# Autodesk Inventor assembly: Tesla_Coul
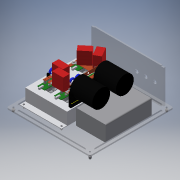
[picture p0: Inventor's stored thumbnail of the model, 180x180]
Saved by Autodesk Inventor 2016 (Build 200138000, 138)
## iProperties
Created: 2018-04-27
Part Number: Tesla_Coul
Document SubType Name: Assembly
Designer: Phil Erle
Author: Phil Erle
## Documents named in this file (43)
- C:\Users\Phil Erle\Desktop\Adrastea\Tesla_Coil.iam
- C:\Users\Phil Erle\Desktop\Adrastea\primary_holder.ipt
- C:\Users\Phil Erle\Desktop\Adrastea\Secondary.ipt
- C:\Users\Phil Erle\Desktop\Adrastea\Seconday_End_Bottom.ipt
- C:\Users\Phil Erle\Desktop\Adrastea\Seconday_End_Top.ipt
- C:\Users\Phil Erle\Desktop\Adrastea\Primary.ipt
- C:\Users\Phil Erle\Desktop\Adrastea\Normteile\Muttern\mutter_din934_m4-10.ipt
- C:\Users\Phil Erle\Desktop\Adrastea\Normteile\Schrauben\M4\Zylinderkopf\din_en_iso_4762_m4x16.ipt
- C:\Users\Phil Erle\Desktop\Adrastea\Coil.ipt
- C:\Users\Phil Erle\Desktop\Adrastea\Main.ipt
- C:\Users\Phil Erle\Desktop\Adrastea\Cap_Platine.ipt
- C:\Users\Phil Erle\Desktop\Adrastea\Strike_Rail.ipt
- C:\Users\Phil Erle\Desktop\Adrastea\Topload stift.ipt
- C:\Users\Phil Erle\Desktop\Adrastea\TopLoad.ipt
- C:\Users\Phil Erle\Desktop\Adrastea\Normteile\Schrauben\M8\din_en_iso_4762_m8x12.ipt
- C:\Users\Phil Erle\Desktop\Adrastea\mid.ipt
- C:\Users\Phil Erle\Desktop\Adrastea\bottom.ipt
- C:\Users\Phil Erle\Desktop\Adrastea\Abstandshalter_10mm.ipt
- C:\Users\Phil Erle\Desktop\Adrastea\M5 Gewindestange.ipt
- C:\Users\Phil Erle\Desktop\Adrastea\Normteile\Muttern\mutter_din934_m5-6.ipt
- C:\Users\Phil Erle\Desktop\Adrastea\Elektronik_Gehäuse.ipt
- C:\Users\Phil Erle\Desktop\Adrastea\GT175DA120U.ipt
- C:\Users\Phil Erle\Desktop\Adrastea\Heatsink.ipt
- C:\Users\Phil Erle\Desktop\Adrastea\Normteile\Schrauben\M3\din_en_iso_4762_m3x8.ipt
- C:\Users\Phil Erle\Desktop\Adrastea\SeitenOben.ipt
- C:\Users\Phil Erle\Desktop\Adrastea\IGBT_Platine.ipt
- C:\Users\Phil Erle\Desktop\Adrastea\Abstandshalter_10mm_M4.ipt
- C:\Users\Phil Erle\Desktop\Adrastea\SeitenUnten.ipt
- C:\Users\Phil Erle\Desktop\Adrastea\Normteile\Schrauben\M3\din_en_iso_4762_m3x10.ipt
- C:\Users\Phil Erle\Desktop\Adrastea\SeitenUntenHinten.ipt
- C:\Users\Phil Erle\Desktop\Adrastea\SeitenUntenVorne.ipt
- C:\Users\Phil Erle\Desktop\Adrastea\Normteile\Muttern\din1587-m5x0_8ricu3.ipt
- C:\Users\Phil Erle\Desktop\Adrastea\Normteile\Muttern\mutter_din934_m3-6.ipt
- C:\Users\Phil Erle\Desktop\Adrastea\Normteile\Schrauben\M4\Zylinderkopf\din_en_iso_4762_m4x6.ipt
- C:\Users\Phil Erle\Desktop\Adrastea\CT.ipt
- C:\Users\Phil Erle\Desktop\Adrastea\Cap_Holder_1.ipt
- C:\Users\Phil Erle\Desktop\Adrastea\CT_Holder.ipt
- C:\Users\Phil Erle\Desktop\Adrastea\Cap.ipt
- C:\Users\Phil Erle\Desktop\Adrastea\CU2.ipt
- C:\Users\Phil Erle\Desktop\Adrastea\CU4.ipt
- C:\Users\Phil Erle\Desktop\Adrastea\Snubber.ipt
- C:\Users\Phil Erle\Desktop\Adrastea\CU5.ipt
- C:\Users\Phil Erle\Desktop\Adrastea\CU6.ipt
## Components (192 placed, 42 different names)
1. primary_holder:1 — Mate:9, Mate:57, Mate:59, Flush:4, Angle:1, Mate:76, Mate:77
2. primary_holder:2 — Mate:8, Mate:48, Mate:49, Mate:50, Mate:51, Flush:6
3. primary_holder:3 — Mate:7, Mate:58, Mate:62, Mate:63, Mate:66, Flush:5
4. primary_holder:4 — Mate:6, Mate:56, Mate:60, Mate:64, Mate:65, Mate:69
5. primary_holder:5 — Mate:5, Mate:55, Mate:61, Flush:3, Mate:74, Mate:75, Mate:230
6. primary_holder:6 — Mate:4, Mate:52, Mate:53, Mate:70, Mate:72, Mate:73
7. Secondary:1 — Mate:3, Mate:11, Mate:12, Mate:13, Mate:79, Mate:80, Flush:7, Mate:81
8. Seconday_End_Bottom:1 — Mate:1, Mate:2, Flush:1, Mate:3, Mate:10, Mate:11, Mate:85, Mate:88
9. Seconday_End_Top:1 — Mate:12, Mate:13, Mate:78, Mate:89, Mate:303
10. Primary:1 — Mate:4, Mate:5, Mate:6, Mate:7, Mate:8, Mate:9, Mate:10, Mate:14, Mate:15, Mate:16, Mate:17, Mate:18, Mate:19, Mate:20, Mate:21, Mate:22, Mate:23, Mate:24, Mate:25, Mate:38, Mate:39, Mate:40, Mate:41, Mate:42, Mate:43, Mate:44, Mate:45, Mate:46, Mate:47, Mate:54, Mate:71, Mate:173, Mate:229, Flush:9, Flush:10, Flush:11, Flush:12
11. mutter_din934_m4-10:1 — Mate:27, Mate:57, Mate:77
12. mutter_din934_m4-10:2 — Mate:28, Mate:62, Mate:63
13. mutter_din934_m4-10:3 — Mate:26, Mate:59, Mate:76
14. mutter_din934_m4-10:4 — Mate:36, Mate:52, Mate:72
15. mutter_din934_m4-10:5 — Mate:30, Mate:48, Mate:50
16. mutter_din934_m4-10:6 — Mate:37, Mate:53, Mate:73
17. mutter_din934_m4-10:7 — Mate:33, Mate:61, Mate:75
18. mutter_din934_m4-10:8 — Mate:34, Mate:55, Mate:74
19. mutter_din934_m4-10:9 — Mate:32, Mate:56, Mate:64
20. mutter_din934_m4-10:10 — Mate:31, Mate:60, Mate:65
21. mutter_din934_m4-10:11 — Mate:35, Mate:49, Mate:51
22. mutter_din934_m4-10:12 — Mate:29, Mate:58, Mate:66
23. din_en_iso_4762_m4x16:1 — Mate:14, Mate:27, Mate:42
24. din_en_iso_4762_m4x16:2 — Mate:15, Mate:26, Mate:39
25. din_en_iso_4762_m4x16:3 — Mate:16, Mate:36, Mate:40
26. din_en_iso_4762_m4x16:4 — Mate:17, Mate:37, Mate:46
27. din_en_iso_4762_m4x16:5 — Mate:24, Mate:35, Mate:45
28. din_en_iso_4762_m4x16:6 — Mate:25, Mate:30, Mate:44
29. din_en_iso_4762_m4x16:7 — Mate:23, Mate:34, Mate:173
30. din_en_iso_4762_m4x16:8 — Mate:22, Mate:33, Mate:47
31. din_en_iso_4762_m4x16:9 — Mate:21, Mate:32, Mate:71
32. din_en_iso_4762_m4x16:10 — Mate:20, Mate:31, Mate:43
33. din_en_iso_4762_m4x16:11 — Mate:18, Mate:29, Mate:38
34. din_en_iso_4762_m4x16:12 — Mate:19, Mate:28, Mate:41
35. Coil:1 — Mate:80, Flush:7
36. Main:1 — Mate:83, Mate:84, Mate:87, Mate:88, Mate:142, Mate:143, Mate:144, Mate:145, Mate:174, Mate:175, Mate:176, Mate:177, Mate:217
37. Cap_Platine:1 — Mate:154, Mate:163, Mate:166
38. Cap_Platine:2 — Mate:155, Mate:160, Mate:161
39. Cap_Platine:3 — Mate:151, Mate:158, Mate:159
40. Cap_Platine:4 — Mate:153, Mate:167, Mate:168
41. Cap_Platine:5 — Mate:150, Mate:156, Mate:157
42. Cap_Platine:6 — Mate:162, Mate:164, Mate:165
43. Strike_Rail:1 — Mate:81, Mate:231, Mate:232
44. Topload stift:1 — Mate:89, Mate:92, Mate:301, Mate:302, Flush:13, Flush:14
45. TopLoad:1 — Mate:92, Mate:303
46. din_en_iso_4762_m8x12:1 — Mate:83, Mate:84, Mate:85
47. mid:1 — Mate:94, Mate:95, Mate:96, Mate:97, Mate:98, Mate:99, Mate:100, Mate:101, Mate:102, Mate:103, Mate:104, Mate:105, Mate:106, Mate:107, Mate:108, Mate:109, Mate:110, Mate:111, Mate:112, Mate:113, Mate:114, Mate:115, Mate:116, Mate:117, Mate:118, Mate:119, Mate:120, Mate:121, Mate:122, Mate:123, Mate:124, Mate:125, Mate:126, Mate:127, Mate:128, Mate:129, Mate:130, Mate:131, Mate:132, Mate:133, Mate:134, Mate:135, Mate:136, Mate:137, Mate:138, Mate:139, Mate:140, Mate:141, Mate:146, Mate:147, Mate:208, Mate:209, Mate:210, Mate:211, Mate:212, Mate:213, Mate:214, Mate:215, Mate:216, Mate:218, Mate:219, Mate:220, Mate:255, Mate:261, Mate:262, Mate:263, Mate:274, Mate:275, Mate:276, Mate:277, Mate:278, Mate:279, Mate:304, Mate:305, Mate:306, Mate:307, Mate:308, Mate:309, Mate:310, Mate:311, Mate:312, Mate:313, Mate:314, Mate:315, Mate:316, Mate:317, Mate:318, Mate:319, Mate:320, Mate:321, Mate:322, Mate:323, Mate:324, Mate:325, Mate:326, Mate:327, Mate:328, Mate:329, Mate:330, Mate:331, Mate:332, Mate:333, Mate:334, Mate:335, Mate:336, Mate:337, Mate:338, Mate:339, Mate:340, Mate:341, Mate:342
48. bottom:1 — Mate:148, Mate:149, Mate:179, Mate:244, Mate:245, Mate:247, Mate:250, Mate:251, Mate:254, Mate:256, Mate:257, Mate:258, Mate:259, Mate:260, Mate:264, Mate:265, Mate:268, Mate:269, Mate:270, Mate:271, Mate:272, Mate:273, Mate:280, Mate:281, Mate:282, Mate:283, Mate:287, Mate:288, Mate:289, Mate:290, Mate:291, Mate:292, Mate:294, Mate:296, Mate:297, Mate:299, Mate:300
49. Abstandshalter_10mm:1 — Mate:94, Mate:138, Mate:168
50. Abstandshalter_10mm:2 — Mate:95, Mate:128, Mate:154, Mate:155, Mate:161
51. Abstandshalter_10mm:3 — Mate:101, Mate:135, Mate:157
52. Abstandshalter_10mm:4 — Mate:97, Mate:121, Mate:160
53. Abstandshalter_10mm:5 — Mate:102, Mate:126, Mate:159
54. Abstandshalter_10mm:6 — Mate:96, Mate:139
55. Abstandshalter_10mm:7 — Mate:115, Mate:137, Mate:167
56. Abstandshalter_10mm:8 — Mate:111, Mate:136
57. Abstandshalter_10mm:9 — Mate:113, Mate:130
58. Abstandshalter_10mm:10 — Mate:116, Mate:140, Mate:150
59. Abstandshalter_10mm:11 — Mate:131, Mate:132
60. Abstandshalter_10mm:12 — Mate:112, Mate:141
61. Abstandshalter_10mm:13 — Mate:114, Mate:133, Mate:156
62. Abstandshalter_10mm:14 — Mate:109, Mate:127
63. Abstandshalter_10mm:15 — Mate:108, Mate:120, Mate:162, Mate:164
64. Abstandshalter_10mm:16 — Mate:104, Mate:122
65. Abstandshalter_10mm:17 — Mate:98, Mate:123
66. Abstandshalter_10mm:18 — Mate:100, Mate:129
67. Abstandshalter_10mm:19 — Mate:99, Mate:134, Mate:158
68. Abstandshalter_10mm:20 — Mate:106, Mate:125
69. Abstandshalter_10mm:21 — Mate:105, Mate:124, Mate:166
70. Abstandshalter_10mm:22 — Mate:103, Mate:118, Mate:153
71. Abstandshalter_10mm:23 — Mate:107, Mate:117, Mate:165
72. Abstandshalter_10mm:24 — Mate:110, Mate:119, Mate:151, Mate:163
73. M5 Gewindestange:1 — Mate:142, Mate:169, Mate:222, Flush:10, Mate:293
74. M5 Gewindestange:2 — Mate:143, Mate:172, Mate:221, Flush:12
75. M5 Gewindestange:3 — Mate:144, Mate:146, Mate:149, Mate:171, Mate:224, Flush:11, Mate:298
76. M5 Gewindestange:4 — Mate:145, Mate:147, Mate:148, Mate:170, Mate:223, Flush:9, Mate:295
77. mutter_din934_m5-6:1 — Mate:172, Mate:177, Mate:226
78. mutter_din934_m5-6:2 — Mate:169, Mate:176, Mate:225
79. mutter_din934_m5-6:3 — Mate:170, Mate:175, Mate:227
80. mutter_din934_m5-6:4 — Mate:171, Mate:174, Mate:228
81. Elektronik_Gehäuse:1 — Mate:283, Mate:284, Mate:285
82. GT175DA120U:1 — Mate:180, Mate:185, Mate:190, Mate:195, Mate:199, Mate:233, Mate:234, Mate:235, Mate:237, Mate:385
83. GT175DA120U:2 — Mate:183, Mate:186, Mate:188, Mate:192, Mate:193, Mate:345, Mate:346, Mate:356, Mate:362, Mate:386
84. GT175DA120U:3 — Mate:181, Mate:184, Mate:189, Mate:194, Mate:197, Mate:358, Mate:359, Mate:360, Mate:369, Mate:384
85. GT175DA120U:4 — Mate:182, Mate:187, Mate:191, Mate:196, Mate:198, Mate:343, Mate:344, Mate:348, Mate:349, Mate:390
86. Heatsink:1 — Mate:179, Mate:180, Mate:181, Mate:182, Mate:183, Mate:200, Mate:201, Mate:202, Mate:203, Mate:204, Mate:205, Mate:206, Mate:207, Mate:266, Mate:267, Mate:377, Mate:379, Mate:381, Mate:383, Mate:392, Mate:395, Mate:398, Mate:399, Mate:400, Mate:401
87. din_en_iso_4762_m3x8:1 — Mate:185, Mate:196, Mate:203
88. din_en_iso_4762_m3x8:2 — Mate:186, Mate:192, Mate:200
89. din_en_iso_4762_m3x8:3 — Mate:187, Mate:198, Mate:204
90. din_en_iso_4762_m3x8:4 — Mate:188, Mate:193, Mate:207
91. din_en_iso_4762_m3x8:5 — Mate:184, Mate:194, Mate:201
92. din_en_iso_4762_m3x8:6 — Mate:189, Mate:195, Mate:205
93. din_en_iso_4762_m3x8:7 — Mate:191, Mate:199, Mate:206
94. din_en_iso_4762_m3x8:8 — Mate:190, Mate:197, Mate:202
95. SeitenOben:1 — Mate:210, Mate:214, Mate:217, Mate:218
96. SeitenOben:2 — Mate:211, Mate:212, Mate:213
97. SeitenOben:3 — Mate:209, Mate:215, Mate:219
98. SeitenOben:4 — Mate:208, Mate:216, Mate:220
99. mutter_din934_m5-6:5 — Mate:221, Mate:226
100. mutter_din934_m5-6:6 — Mate:224, Mate:228
101. mutter_din934_m5-6:7 — Mate:223, Mate:227, Mate:229
102. mutter_din934_m5-6:8 — Mate:222, Mate:225
103. IGBT_Platine:1 — Mate:233, Mate:236, Mate:239, Mate:240, Mate:241, Mate:286, Mate:389
104. IGBT_Platine:2 — Mate:356, Mate:363, Mate:364, Mate:365, Mate:367, Mate:368, Mate:387
105. IGBT_Platine:3 — Mate:369, Mate:371, Mate:372, Mate:373, Mate:375, Mate:388
106. IGBT_Platine:4 — Mate:349, Mate:350, Mate:351, Mate:352, Mate:354, Mate:355, Mate:391
107. Abstandshalter_10mm_M4:1 — Mate:235, Mate:240, Mate:441
108. Abstandshalter_10mm_M4:2 — Mate:234, Mate:236, Mate:239, Mate:440
109. Abstandshalter_10mm_M4:4 — Mate:237, Mate:241, Mate:286, Mate:434, Mate:451
110. SeitenUnten:1 — Mate:244, Mate:247, Mate:254, Mate:255
111. SeitenUnten:3 — Mate:245, Mate:250, Mate:251
112. din_en_iso_4762_m3x10:1 — Mate:317, Mate:331
113. din_en_iso_4762_m3x10:2 — Mate:256, Mate:265, Mate:266, Mate:380
114. din_en_iso_4762_m3x10:3 — Mate:316, Mate:328
115. din_en_iso_4762_m3x10:4 — Mate:321, Mate:327
116. din_en_iso_4762_m3x10:5 — Mate:263, Mate:338
117. din_en_iso_4762_m3x10:6 — Mate:319, Mate:334
118. din_en_iso_4762_m3x10:7 — Mate:262, Mate:341
119. din_en_iso_4762_m3x10:8 — Mate:318, Mate:323
120. din_en_iso_4762_m3x10:9 — Mate:320, Mate:326
121. din_en_iso_4762_m3x10:10 — Mate:315, Mate:329
122. din_en_iso_4762_m3x10:11 — Mate:311, Mate:339
123. din_en_iso_4762_m3x10:12 — Mate:310, Mate:325
124. din_en_iso_4762_m3x10:13 — Mate:308, Mate:324
125. din_en_iso_4762_m3x10:14 — Mate:309, Mate:336
126. din_en_iso_4762_m3x10:15 — Mate:306, Mate:330
127. din_en_iso_4762_m3x10:16 — Mate:312, Mate:335
128. din_en_iso_4762_m3x10:17 — Mate:307, Mate:332
129. din_en_iso_4762_m3x10:18 — Mate:313, Mate:333
130. din_en_iso_4762_m3x10:19 — Mate:314, Mate:342
131. din_en_iso_4762_m3x10:20 — Mate:261, Mate:337
132. din_en_iso_4762_m3x10:21 — Mate:271, Mate:280, Mate:284
133. din_en_iso_4762_m3x10:22 — Mate:258, Mate:269
134. din_en_iso_4762_m3x10:23 — Mate:272, Mate:282, Mate:285
135. din_en_iso_4762_m3x10:24 — Mate:257, Mate:268, Mate:378
136. din_en_iso_4762_m3x10:25 — Mate:304, Mate:322
137. din_en_iso_4762_m3x10:26 — Mate:274, Mate:278
138. din_en_iso_4762_m3x10:27 — Mate:273, Mate:281
139. din_en_iso_4762_m3x10:28 — Mate:259, Mate:270, Mate:382
140. din_en_iso_4762_m3x10:29 — Mate:305, Mate:340
141. din_en_iso_4762_m3x10:30 — Mate:275, Mate:277
142. din_en_iso_4762_m3x10:31 — Mate:276, Mate:279
143. din_en_iso_4762_m3x10:32 — Mate:260, Mate:264, Mate:267, Mate:376
144. SeitenUntenHinten:1 — Mate:287, Mate:288, Mate:289
145. SeitenUntenVorne:1 — Mate:290, Mate:291, Mate:292
146. din1587-m5x0_8ricu3:1 — Mate:293, Mate:294
147. din1587-m5x0_8ricu3:2 — Mate:295, Mate:296
148. din1587-m5x0_8ricu3:3 — Mate:297, Mate:300
149. din1587-m5x0_8ricu3:4 — Mate:298, Mate:299
150. mutter_din934_m5-6:9 — Mate:301, Flush:14
151. mutter_din934_m5-6:10 — Mate:302, Flush:13
152. Abstandshalter_10mm_M4:5 — Mate:344, Mate:352, Mate:422, Mate:437
153. Abstandshalter_10mm_M4:6 — Mate:346, Mate:363, Mate:368, Mate:420
154. Abstandshalter_10mm_M4:7 — Mate:345, Mate:365, Mate:367, Mate:421
155. Abstandshalter_10mm_M4:8 — Mate:343, Mate:350, Mate:355, Mate:442
156. Abstandshalter_10mm_M4:10 — Mate:348, Mate:351, Mate:354
157. Abstandshalter_10mm_M4:11 — Mate:359, Mate:371
158. Abstandshalter_10mm_M4:12 — Mate:360, Mate:372, Mate:375, Mate:450
159. Abstandshalter_10mm_M4:14 — Mate:358, Mate:373, Mate:412, Mate:416
160. Abstandshalter_10mm_M4:16 — Mate:362, Mate:364, Mate:417
161. mutter_din934_m3-6:1 — Mate:376, Mate:377
162. mutter_din934_m3-6:2 — Mate:380, Mate:381
163. mutter_din934_m3-6:3 — Mate:378, Mate:379
164. mutter_din934_m3-6:4 — Mate:382, Mate:383
165. din_en_iso_4762_m4x6:1 — Mate:384, Mate:388
166. din_en_iso_4762_m4x6:2 — Mate:385, Mate:389
167. din_en_iso_4762_m4x6:3 — Mate:386, Mate:387
168. din_en_iso_4762_m4x6:4 — Mate:390, Mate:391
169. CT:1 — Mate:394, Flush:15
170. CT:2 — Mate:393, Flush:16
171. CT:3 — Mate:396, Flush:17
172. CT:4 — Mate:397, Flush:18
173. Cap_Holder_1:1 — Mate:399, Mate:400, Mate:407
174. Cap_Holder_1:2 — Mate:392, Mate:401, Mate:406
175. CT_Holder:1 — Mate:396, Mate:397, Flush:17, Flush:18, Mate:398
176. CT_Holder:2 — Mate:393, Mate:394, Flush:15, Flush:16, Mate:395
177. Cap:1 — Mate:407, Mate:415, Mate:431
178. Cap:2 — Mate:406, Mate:414, Mate:429, Mate:430
179. CU2:1 — Mate:412, Mate:414, Mate:415, Mate:418, Mate:419, Mate:438, Mate:439, Mate:443, Mate:444
180. din_en_iso_4762_m4x6:5 — Mate:416, Mate:419, Mate:443
181. din_en_iso_4762_m4x6:6 — Mate:421
182. din_en_iso_4762_m4x6:7 — Mate:422, Mate:445
183. din_en_iso_4762_m4x6:8 — Mate:420
184. din_en_iso_4762_m4x6:9 — Mate:417, Mate:418, Mate:444
185. CU4:1 — Mate:429, Mate:430, Mate:431
186. Snubber:1 — Mate:446, Mate:449
187. Snubber:2 — Mate:439
188. Snubber:3 — Mate:447, Mate:452
189. Snubber:4 — Mate:438
190. CU5:1 — Mate:434, Mate:450, Mate:451
191. CU5:2 — Mate:437, Mate:445
192. CU6:1 — Mate:440, Mate:441, Mate:442, Mate:446, Mate:447, Mate:449, Mate:452
## Relationships (429: Mate 410, Flush 16, Angle 3)
- Mate:1: Seconday_End_Bottom:1
- Mate:2: Seconday_End_Bottom:1
- Flush:1: Seconday_End_Bottom:1
- Mate:3: Secondary:1 ↔ Seconday_End_Bottom:1
- Mate:4: primary_holder:6 ↔ Primary:1
- Mate:5: primary_holder:5 ↔ Primary:1
- Mate:6: primary_holder:4 ↔ Primary:1
- Mate:7: primary_holder:3 ↔ Primary:1
- Mate:8: primary_holder:2 ↔ Primary:1
- Mate:9: primary_holder:1 ↔ Primary:1
- Mate:10: Seconday_End_Bottom:1 ↔ Primary:1
- Mate:11: Secondary:1 ↔ Seconday_End_Bottom:1
- Mate:12: Secondary:1 ↔ Seconday_End_Top:1
- Mate:13: Secondary:1 ↔ Seconday_End_Top:1
- Mate:14: Primary:1 ↔ din_en_iso_4762_m4x16:1
- Mate:15: Primary:1 ↔ din_en_iso_4762_m4x16:2
- Mate:16: Primary:1 ↔ din_en_iso_4762_m4x16:3
- Mate:17: Primary:1 ↔ din_en_iso_4762_m4x16:4
- Mate:18: Primary:1 ↔ din_en_iso_4762_m4x16:11
- Mate:19: Primary:1 ↔ din_en_iso_4762_m4x16:12
- Mate:20: Primary:1 ↔ din_en_iso_4762_m4x16:10
- Mate:21: Primary:1 ↔ din_en_iso_4762_m4x16:9
- Mate:22: Primary:1 ↔ din_en_iso_4762_m4x16:8
- Mate:23: Primary:1 ↔ din_en_iso_4762_m4x16:7
- Mate:24: Primary:1 ↔ din_en_iso_4762_m4x16:5
- Mate:25: Primary:1 ↔ din_en_iso_4762_m4x16:6
- Mate:26: mutter_din934_m4-10:3 ↔ din_en_iso_4762_m4x16:2
- Mate:27: mutter_din934_m4-10:1 ↔ din_en_iso_4762_m4x16:1
- Mate:28: mutter_din934_m4-10:2 ↔ din_en_iso_4762_m4x16:12
- Mate:29: mutter_din934_m4-10:12 ↔ din_en_iso_4762_m4x16:11
- Mate:30: mutter_din934_m4-10:5 ↔ din_en_iso_4762_m4x16:6
- Mate:31: mutter_din934_m4-10:10 ↔ din_en_iso_4762_m4x16:10
- Mate:32: mutter_din934_m4-10:9 ↔ din_en_iso_4762_m4x16:9
- Mate:33: mutter_din934_m4-10:7 ↔ din_en_iso_4762_m4x16:8
- Mate:34: mutter_din934_m4-10:8 ↔ din_en_iso_4762_m4x16:7
- Mate:35: mutter_din934_m4-10:11 ↔ din_en_iso_4762_m4x16:5
- Mate:36: mutter_din934_m4-10:4 ↔ din_en_iso_4762_m4x16:3
- Mate:37: mutter_din934_m4-10:6 ↔ din_en_iso_4762_m4x16:4
- Mate:38: Primary:1 ↔ din_en_iso_4762_m4x16:11
- Mate:39: Primary:1 ↔ din_en_iso_4762_m4x16:2
- Mate:40: Primary:1 ↔ din_en_iso_4762_m4x16:3
- Mate:41: Primary:1 ↔ din_en_iso_4762_m4x16:12
- Mate:42: Primary:1 ↔ din_en_iso_4762_m4x16:1
- Mate:43: Primary:1 ↔ din_en_iso_4762_m4x16:10
- Mate:44: Primary:1 ↔ din_en_iso_4762_m4x16:6
- Mate:45: Primary:1 ↔ din_en_iso_4762_m4x16:5
- Mate:46: Primary:1 ↔ din_en_iso_4762_m4x16:4
- Mate:47: Primary:1 ↔ din_en_iso_4762_m4x16:8
- Mate:48: primary_holder:2 ↔ mutter_din934_m4-10:5
- Mate:49: primary_holder:2 ↔ mutter_din934_m4-10:11
- Mate:50: primary_holder:2 ↔ mutter_din934_m4-10:5
- Mate:51: primary_holder:2 ↔ mutter_din934_m4-10:11
- Mate:52: primary_holder:6 ↔ mutter_din934_m4-10:4
- Mate:53: primary_holder:6 ↔ mutter_din934_m4-10:6
- Mate:54: Primary:1
- Mate:55: primary_holder:5 ↔ mutter_din934_m4-10:8
- Mate:56: primary_holder:4 ↔ mutter_din934_m4-10:9
- Mate:57: primary_holder:1 ↔ mutter_din934_m4-10:1
- Mate:58: primary_holder:3 ↔ mutter_din934_m4-10:12
- Mate:59: primary_holder:1 ↔ mutter_din934_m4-10:3
- Mate:60: primary_holder:4 ↔ mutter_din934_m4-10:10
- Mate:61: primary_holder:5 ↔ mutter_din934_m4-10:7
- Mate:62: primary_holder:3 ↔ mutter_din934_m4-10:2
- Mate:63: primary_holder:3 ↔ mutter_din934_m4-10:2
- Mate:64: primary_holder:4 ↔ mutter_din934_m4-10:9
- Mate:65: primary_holder:4 ↔ mutter_din934_m4-10:10
- Mate:66: primary_holder:3 ↔ mutter_din934_m4-10:12
- Flush:3 (2.5 mm): primary_holder:5
- Flush:4 (2.5 mm): primary_holder:1
- Mate:67
- Angle:1 (60 deg): primary_holder:1
- Flush:5 (2.5 mm): primary_holder:3
- Flush:6 (2.5 mm): primary_holder:2
- Mate:68
- Angle:2 (-60 deg)
- Mate:69 (-2.5 mm): primary_holder:4
- Mate:70 (-2.5 mm): primary_holder:6
- Mate:71: Primary:1 ↔ din_en_iso_4762_m4x16:9
- Mate:72: primary_holder:6 ↔ mutter_din934_m4-10:4
- Mate:73: primary_holder:6 ↔ mutter_din934_m4-10:6
- Mate:74: primary_holder:5 ↔ mutter_din934_m4-10:8
- Mate:75: primary_holder:5 ↔ mutter_din934_m4-10:7
- Mate:76: primary_holder:1 ↔ mutter_din934_m4-10:3
- Mate:77: primary_holder:1 ↔ mutter_din934_m4-10:1
- Mate:78: Seconday_End_Top:1
- Mate:79: Secondary:1
- Mate:80: Secondary:1 ↔ Coil:1
- Flush:7 (-50 mm): Secondary:1 ↔ Coil:1
- Mate:81: Secondary:1 ↔ Strike_Rail:1
- Mate:83: Main:1 ↔ din_en_iso_4762_m8x12:1
- Mate:84: Main:1 ↔ din_en_iso_4762_m8x12:1
- Mate:85: Seconday_End_Bottom:1 ↔ din_en_iso_4762_m8x12:1
- Mate:87: Main:1
- Mate:88: Seconday_End_Bottom:1 ↔ Main:1
- Mate:89: Seconday_End_Top:1 ↔ Topload stift:1
- Mate:92: Topload stift:1 ↔ TopLoad:1
- Mate:94: mid:1 ↔ Abstandshalter_10mm:1
- Mate:95: mid:1 ↔ Abstandshalter_10mm:2
- Mate:96: mid:1 ↔ Abstandshalter_10mm:6
- Mate:97: mid:1 ↔ Abstandshalter_10mm:4
- Mate:98: mid:1 ↔ Abstandshalter_10mm:17
- Mate:99: mid:1 ↔ Abstandshalter_10mm:19
- Mate:100: mid:1 ↔ Abstandshalter_10mm:18
- Mate:101: mid:1 ↔ Abstandshalter_10mm:3
- Mate:102: mid:1 ↔ Abstandshalter_10mm:5
- Mate:103: mid:1 ↔ Abstandshalter_10mm:22
- Mate:104: mid:1 ↔ Abstandshalter_10mm:16
- Mate:105: mid:1 ↔ Abstandshalter_10mm:21
- Mate:106: mid:1 ↔ Abstandshalter_10mm:20
- Mate:107: mid:1 ↔ Abstandshalter_10mm:23
- Mate:108: mid:1 ↔ Abstandshalter_10mm:15
- Mate:109: mid:1 ↔ Abstandshalter_10mm:14
- Mate:110: mid:1 ↔ Abstandshalter_10mm:24
- Mate:111: mid:1 ↔ Abstandshalter_10mm:8
- Mate:112: mid:1 ↔ Abstandshalter_10mm:12
- Mate:113: mid:1 ↔ Abstandshalter_10mm:9
- Mate:114: mid:1 ↔ Abstandshalter_10mm:13
- Mate:115: mid:1 ↔ Abstandshalter_10mm:7
- Mate:116: mid:1 ↔ Abstandshalter_10mm:10
- Mate:117: mid:1 ↔ Abstandshalter_10mm:23
- Mate:118: mid:1 ↔ Abstandshalter_10mm:22
- Mate:119: mid:1 ↔ Abstandshalter_10mm:24
- Mate:120: mid:1 ↔ Abstandshalter_10mm:15
- Mate:121: mid:1 ↔ Abstandshalter_10mm:4
- Mate:122: mid:1 ↔ Abstandshalter_10mm:16
- Mate:123: mid:1 ↔ Abstandshalter_10mm:17
- Mate:124: mid:1 ↔ Abstandshalter_10mm:21
- Mate:125: mid:1 ↔ Abstandshalter_10mm:20
- Mate:126: mid:1 ↔ Abstandshalter_10mm:5
- Mate:127: mid:1 ↔ Abstandshalter_10mm:14
- Mate:128: mid:1 ↔ Abstandshalter_10mm:2
- Mate:129: mid:1 ↔ Abstandshalter_10mm:18
- Mate:130: mid:1 ↔ Abstandshalter_10mm:9
- Mate:131: mid:1 ↔ Abstandshalter_10mm:11
- Mate:132: mid:1 ↔ Abstandshalter_10mm:11
- Mate:133: mid:1 ↔ Abstandshalter_10mm:13
- Mate:134: mid:1 ↔ Abstandshalter_10mm:19
- Mate:135: mid:1 ↔ Abstandshalter_10mm:3
- Mate:136: mid:1 ↔ Abstandshalter_10mm:8
- Mate:137: mid:1 ↔ Abstandshalter_10mm:7
- Mate:138: mid:1 ↔ Abstandshalter_10mm:1
- Mate:139: mid:1 ↔ Abstandshalter_10mm:6
- Mate:140: mid:1 ↔ Abstandshalter_10mm:10
- Mate:141: mid:1 ↔ Abstandshalter_10mm:12
- Mate:142: Main:1 ↔ M5 Gewindestange:1
- Mate:143: Main:1 ↔ M5 Gewindestange:2
- Mate:144: Main:1 ↔ M5 Gewindestange:3
- Mate:145: Main:1 ↔ M5 Gewindestange:4
- Mate:146: mid:1 ↔ M5 Gewindestange:3
- Mate:147: mid:1 ↔ M5 Gewindestange:4
- Mate:148: bottom:1 ↔ M5 Gewindestange:4
- Mate:149: bottom:1 ↔ M5 Gewindestange:3
- Mate:150: Cap_Platine:5 ↔ Abstandshalter_10mm:10
- Mate:151: Cap_Platine:3 ↔ Abstandshalter_10mm:24
- Mate:153: Cap_Platine:4 ↔ Abstandshalter_10mm:22
- Mate:154: Cap_Platine:1 ↔ Abstandshalter_10mm:2
- Mate:155: Cap_Platine:2 ↔ Abstandshalter_10mm:2
- Mate:156: Cap_Platine:5 ↔ Abstandshalter_10mm:13
- Mate:157: Cap_Platine:5 ↔ Abstandshalter_10mm:3
- Mate:158: Cap_Platine:3 ↔ Abstandshalter_10mm:19
- Mate:159: Cap_Platine:3 ↔ Abstandshalter_10mm:5
- Mate:160: Cap_Platine:2 ↔ Abstandshalter_10mm:4
- Mate:161: Cap_Platine:2 ↔ Abstandshalter_10mm:2
- Mate:162: Cap_Platine:6 ↔ Abstandshalter_10mm:15
- Mate:163: Cap_Platine:1 ↔ Abstandshalter_10mm:24
- Mate:164: Cap_Platine:6 ↔ Abstandshalter_10mm:15
- Mate:165: Cap_Platine:6 ↔ Abstandshalter_10mm:23
- Mate:166: Cap_Platine:1 ↔ Abstandshalter_10mm:21
- Mate:167: Cap_Platine:4 ↔ Abstandshalter_10mm:7
- Mate:168: Cap_Platine:4 ↔ Abstandshalter_10mm:1
- Mate:169: M5 Gewindestange:1 ↔ mutter_din934_m5-6:2
- Mate:170: M5 Gewindestange:4 ↔ mutter_din934_m5-6:3
- Mate:171: M5 Gewindestange:3 ↔ mutter_din934_m5-6:4
- Mate:172: M5 Gewindestange:2 ↔ mutter_din934_m5-6:1
- Mate:173: Primary:1 ↔ din_en_iso_4762_m4x16:7
- Mate:174: Main:1 ↔ mutter_din934_m5-6:4
- Mate:175: Main:1 ↔ mutter_din934_m5-6:3
- Mate:176: Main:1 ↔ mutter_din934_m5-6:2
- Mate:177: Main:1 ↔ mutter_din934_m5-6:1
- Mate:179: bottom:1 ↔ Heatsink:1
- Mate:180: GT175DA120U:1 ↔ Heatsink:1
- Mate:181: GT175DA120U:3 ↔ Heatsink:1
- Mate:182: GT175DA120U:4 ↔ Heatsink:1
- Mate:183: GT175DA120U:2 ↔ Heatsink:1
- Mate:184: GT175DA120U:3 ↔ din_en_iso_4762_m3x8:5
- Mate:185: GT175DA120U:1 ↔ din_en_iso_4762_m3x8:1
- Mate:186: GT175DA120U:2 ↔ din_en_iso_4762_m3x8:2
- Mate:187: GT175DA120U:4 ↔ din_en_iso_4762_m3x8:3
- Mate:188: GT175DA120U:2 ↔ din_en_iso_4762_m3x8:4
- Mate:189: GT175DA120U:3 ↔ din_en_iso_4762_m3x8:6
- Mate:190: GT175DA120U:1 ↔ din_en_iso_4762_m3x8:8
- Mate:191: GT175DA120U:4 ↔ din_en_iso_4762_m3x8:7
- Mate:192: GT175DA120U:2 ↔ din_en_iso_4762_m3x8:2
- Mate:193: GT175DA120U:2 ↔ din_en_iso_4762_m3x8:4
- Mate:194: GT175DA120U:3 ↔ din_en_iso_4762_m3x8:5
- Mate:195: GT175DA120U:1 ↔ din_en_iso_4762_m3x8:6
- Mate:196: GT175DA120U:4 ↔ din_en_iso_4762_m3x8:1
- Mate:197: GT175DA120U:3 ↔ din_en_iso_4762_m3x8:8
- Mate:198: GT175DA120U:4 ↔ din_en_iso_4762_m3x8:3
- Mate:199: GT175DA120U:1 ↔ din_en_iso_4762_m3x8:7
- Mate:200: Heatsink:1 ↔ din_en_iso_4762_m3x8:2
- Mate:201: Heatsink:1 ↔ din_en_iso_4762_m3x8:5
- Mate:202: Heatsink:1 ↔ din_en_iso_4762_m3x8:8
- Mate:203: Heatsink:1 ↔ din_en_iso_4762_m3x8:1
- Mate:204: Heatsink:1 ↔ din_en_iso_4762_m3x8:3
- Mate:205: Heatsink:1 ↔ din_en_iso_4762_m3x8:6
- Mate:206: Heatsink:1 ↔ din_en_iso_4762_m3x8:7
- Mate:207: Heatsink:1 ↔ din_en_iso_4762_m3x8:4
- Mate:208: mid:1 ↔ SeitenOben:4
- Mate:209: mid:1 ↔ SeitenOben:3
- Mate:210: mid:1 ↔ SeitenOben:1
- Mate:211: mid:1 ↔ SeitenOben:2
- Mate:212: mid:1 ↔ SeitenOben:2
- Mate:213: mid:1 ↔ SeitenOben:2
- Mate:214: mid:1 ↔ SeitenOben:1
- Mate:215: mid:1 ↔ SeitenOben:3
- Mate:216: mid:1 ↔ SeitenOben:4
- Mate:217: Main:1 ↔ SeitenOben:1
- Mate:218: mid:1 ↔ SeitenOben:1
- Mate:219: mid:1 ↔ SeitenOben:3
- Mate:220: mid:1 ↔ SeitenOben:4
- Mate:221: M5 Gewindestange:2 ↔ mutter_din934_m5-6:5
- Mate:222: M5 Gewindestange:1 ↔ mutter_din934_m5-6:8
- Mate:223: M5 Gewindestange:4 ↔ mutter_din934_m5-6:7
- Mate:224: M5 Gewindestange:3 ↔ mutter_din934_m5-6:6
- Mate:225 (45 mm): mutter_din934_m5-6:2 ↔ mutter_din934_m5-6:8
- Mate:226 (45 mm): mutter_din934_m5-6:1 ↔ mutter_din934_m5-6:5
- Mate:227 (45 mm): mutter_din934_m5-6:3 ↔ mutter_din934_m5-6:7
- Mate:228 (45 mm): mutter_din934_m5-6:4 ↔ mutter_din934_m5-6:6
- Mate:229: Primary:1 ↔ mutter_din934_m5-6:7
- Flush:9 (-25 mm): Primary:1 ↔ M5 Gewindestange:4
- Flush:10 (-25 mm): Primary:1 ↔ M5 Gewindestange:1
- Flush:11 (-25 mm): Primary:1 ↔ M5 Gewindestange:3
- Flush:12 (-25 mm): Primary:1 ↔ M5 Gewindestange:2
- Mate:230: primary_holder:5
- Angle:3 (0 deg)
- Mate:231: Strike_Rail:1
- Mate:232: Strike_Rail:1
- Mate:233: GT175DA120U:1 ↔ IGBT_Platine:1
- Mate:234: GT175DA120U:1 ↔ Abstandshalter_10mm_M4:2
- Mate:235: GT175DA120U:1 ↔ Abstandshalter_10mm_M4:1
- Mate:236: IGBT_Platine:1 ↔ Abstandshalter_10mm_M4:2
- Mate:237: GT175DA120U:1 ↔ Abstandshalter_10mm_M4:4
- Mate:239: IGBT_Platine:1 ↔ Abstandshalter_10mm_M4:2
- Mate:240: IGBT_Platine:1 ↔ Abstandshalter_10mm_M4:1
- Mate:241: IGBT_Platine:1 ↔ Abstandshalter_10mm_M4:4
- Mate:244: bottom:1 ↔ SeitenUnten:1
- Mate:245: bottom:1 ↔ SeitenUnten:3
- Mate:247: bottom:1 ↔ SeitenUnten:1
- Mate:250: bottom:1 ↔ SeitenUnten:3
- Mate:251: bottom:1 ↔ SeitenUnten:3
- Mate:254: bottom:1 ↔ SeitenUnten:1
- Mate:255: mid:1 ↔ SeitenUnten:1
- Mate:256: bottom:1 ↔ din_en_iso_4762_m3x10:2
- Mate:257: bottom:1 ↔ din_en_iso_4762_m3x10:24
- Mate:258: bottom:1 ↔ din_en_iso_4762_m3x10:22
- Mate:259: bottom:1 ↔ din_en_iso_4762_m3x10:28
- Mate:260: bottom:1 ↔ din_en_iso_4762_m3x10:32
- Mate:261: mid:1 ↔ din_en_iso_4762_m3x10:20
- Mate:262: mid:1 ↔ din_en_iso_4762_m3x10:7
- Mate:263: mid:1 ↔ din_en_iso_4762_m3x10:5
- Mate:264: bottom:1 ↔ din_en_iso_4762_m3x10:32
- Mate:265: bottom:1 ↔ din_en_iso_4762_m3x10:2
- Mate:266: Heatsink:1 ↔ din_en_iso_4762_m3x10:2
- Mate:267: Heatsink:1 ↔ din_en_iso_4762_m3x10:32
- Mate:268: bottom:1 ↔ din_en_iso_4762_m3x10:24
- Mate:269: bottom:1 ↔ din_en_iso_4762_m3x10:22
- Mate:270: bottom:1 ↔ din_en_iso_4762_m3x10:28
- Mate:271: bottom:1 ↔ din_en_iso_4762_m3x10:21
- Mate:272: bottom:1 ↔ din_en_iso_4762_m3x10:23
- Mate:273: bottom:1 ↔ din_en_iso_4762_m3x10:27
- Mate:274: mid:1 ↔ din_en_iso_4762_m3x10:26
- Mate:275: mid:1 ↔ din_en_iso_4762_m3x10:30
- Mate:276: mid:1 ↔ din_en_iso_4762_m3x10:31
- Mate:277: mid:1 ↔ din_en_iso_4762_m3x10:30
- Mate:278: mid:1 ↔ din_en_iso_4762_m3x10:26
- Mate:279: mid:1 ↔ din_en_iso_4762_m3x10:31
- Mate:280: bottom:1 ↔ din_en_iso_4762_m3x10:21
- Mate:281: bottom:1 ↔ din_en_iso_4762_m3x10:27
- Mate:282: bottom:1 ↔ din_en_iso_4762_m3x10:23
- Mate:283: bottom:1 ↔ Elektronik_Gehäuse:1
- Mate:284: Elektronik_Gehäuse:1 ↔ din_en_iso_4762_m3x10:21
- Mate:285: Elektronik_Gehäuse:1 ↔ din_en_iso_4762_m3x10:23
- Mate:286: IGBT_Platine:1 ↔ Abstandshalter_10mm_M4:4
- Mate:287: bottom:1 ↔ SeitenUntenHinten:1
- Mate:288: bottom:1 ↔ SeitenUntenHinten:1
- Mate:289: bottom:1 ↔ SeitenUntenHinten:1
- Mate:290: bottom:1 ↔ SeitenUntenVorne:1
- Mate:291: bottom:1 ↔ SeitenUntenVorne:1
- Mate:292: bottom:1 ↔ SeitenUntenVorne:1
- Mate:293: M5 Gewindestange:1 ↔ din1587-m5x0_8ricu3:1
- Mate:294: bottom:1 ↔ din1587-m5x0_8ricu3:1
- Mate:295: M5 Gewindestange:4 ↔ din1587-m5x0_8ricu3:2
- Mate:296: bottom:1 ↔ din1587-m5x0_8ricu3:2
- Mate:297: bottom:1 ↔ din1587-m5x0_8ricu3:3
- Mate:298: M5 Gewindestange:3 ↔ din1587-m5x0_8ricu3:4
- Mate:299: bottom:1 ↔ din1587-m5x0_8ricu3:4
- Mate:300: bottom:1 ↔ din1587-m5x0_8ricu3:3
- Mate:301: Topload stift:1 ↔ mutter_din934_m5-6:9
- Mate:302: Topload stift:1 ↔ mutter_din934_m5-6:10
- Flush:13: Topload stift:1 ↔ mutter_din934_m5-6:10
- Flush:14: Topload stift:1 ↔ mutter_din934_m5-6:9
- Mate:303 (150 mm): Seconday_End_Top:1 ↔ TopLoad:1
- Mate:304: mid:1 ↔ din_en_iso_4762_m3x10:25
- Mate:305: mid:1 ↔ din_en_iso_4762_m3x10:29
- Mate:306: mid:1 ↔ din_en_iso_4762_m3x10:15
- Mate:307: mid:1 ↔ din_en_iso_4762_m3x10:17
- Mate:308: mid:1 ↔ din_en_iso_4762_m3x10:13
- Mate:309: mid:1 ↔ din_en_iso_4762_m3x10:14
- Mate:310: mid:1 ↔ din_en_iso_4762_m3x10:12
- Mate:311: mid:1 ↔ din_en_iso_4762_m3x10:11
- Mate:312: mid:1 ↔ din_en_iso_4762_m3x10:16
- Mate:313: mid:1 ↔ din_en_iso_4762_m3x10:18
- Mate:314: mid:1 ↔ din_en_iso_4762_m3x10:19
- Mate:315: mid:1 ↔ din_en_iso_4762_m3x10:10
- Mate:316: mid:1 ↔ din_en_iso_4762_m3x10:3
- Mate:317: mid:1 ↔ din_en_iso_4762_m3x10:1
- Mate:318: mid:1 ↔ din_en_iso_4762_m3x10:8
- Mate:319: mid:1 ↔ din_en_iso_4762_m3x10:6
- Mate:320: mid:1 ↔ din_en_iso_4762_m3x10:9
- Mate:321: mid:1 ↔ din_en_iso_4762_m3x10:4
- Mate:322: mid:1 ↔ din_en_iso_4762_m3x10:25
- Mate:323: mid:1 ↔ din_en_iso_4762_m3x10:8
- Mate:324: mid:1 ↔ din_en_iso_4762_m3x10:13
- Mate:325: mid:1 ↔ din_en_iso_4762_m3x10:12
- Mate:326: mid:1 ↔ din_en_iso_4762_m3x10:9
- Mate:327: mid:1 ↔ din_en_iso_4762_m3x10:4
- Mate:328: mid:1 ↔ din_en_iso_4762_m3x10:3
- Mate:329: mid:1 ↔ din_en_iso_4762_m3x10:10
- Mate:330: mid:1 ↔ din_en_iso_4762_m3x10:15
- Mate:331: mid:1 ↔ din_en_iso_4762_m3x10:1
- Mate:332: mid:1 ↔ din_en_iso_4762_m3x10:17
- Mate:333: mid:1 ↔ din_en_iso_4762_m3x10:18
- Mate:334: mid:1 ↔ din_en_iso_4762_m3x10:6
- Mate:335: mid:1 ↔ din_en_iso_4762_m3x10:16
- Mate:336: mid:1 ↔ din_en_iso_4762_m3x10:14
- Mate:337: mid:1 ↔ din_en_iso_4762_m3x10:20
- Mate:338: mid:1 ↔ din_en_iso_4762_m3x10:5
- Mate:339: mid:1 ↔ din_en_iso_4762_m3x10:11
- Mate:340: mid:1 ↔ din_en_iso_4762_m3x10:29
- Mate:341: mid:1 ↔ din_en_iso_4762_m3x10:7
- Mate:342: mid:1 ↔ din_en_iso_4762_m3x10:19
- Mate:343: GT175DA120U:4 ↔ Abstandshalter_10mm_M4:8
- Mate:344: GT175DA120U:4 ↔ Abstandshalter_10mm_M4:5
- Mate:345: GT175DA120U:2 ↔ Abstandshalter_10mm_M4:7
- Mate:346: GT175DA120U:2 ↔ Abstandshalter_10mm_M4:6
- Mate:348: GT175DA120U:4 ↔ Abstandshalter_10mm_M4:10
- Mate:349: GT175DA120U:4 ↔ IGBT_Platine:4
- Mate:350: IGBT_Platine:4 ↔ Abstandshalter_10mm_M4:8
- Mate:351: IGBT_Platine:4 ↔ Abstandshalter_10mm_M4:10
- Mate:352: IGBT_Platine:4 ↔ Abstandshalter_10mm_M4:5
- Mate:354: IGBT_Platine:4 ↔ Abstandshalter_10mm_M4:10
- Mate:355: IGBT_Platine:4 ↔ Abstandshalter_10mm_M4:8
- Mate:356: GT175DA120U:2 ↔ IGBT_Platine:2
- Mate:358: GT175DA120U:3 ↔ Abstandshalter_10mm_M4:14
- Mate:359: GT175DA120U:3 ↔ Abstandshalter_10mm_M4:11
- Mate:360: GT175DA120U:3 ↔ Abstandshalter_10mm_M4:12
- Mate:362: GT175DA120U:2 ↔ Abstandshalter_10mm_M4:16
- Mate:363: IGBT_Platine:2 ↔ Abstandshalter_10mm_M4:6
- Mate:364: IGBT_Platine:2 ↔ Abstandshalter_10mm_M4:16
- Mate:365: IGBT_Platine:2 ↔ Abstandshalter_10mm_M4:7
- Mate:367: IGBT_Platine:2 ↔ Abstandshalter_10mm_M4:7
- Mate:368: IGBT_Platine:2 ↔ Abstandshalter_10mm_M4:6
- Mate:369: GT175DA120U:3 ↔ IGBT_Platine:3
- Mate:371: IGBT_Platine:3 ↔ Abstandshalter_10mm_M4:11
- Mate:372: IGBT_Platine:3 ↔ Abstandshalter_10mm_M4:12
- Mate:373: IGBT_Platine:3 ↔ Abstandshalter_10mm_M4:14
- Mate:375: IGBT_Platine:3 ↔ Abstandshalter_10mm_M4:12
- Mate:376: din_en_iso_4762_m3x10:32 ↔ mutter_din934_m3-6:1
- Mate:377: Heatsink:1 ↔ mutter_din934_m3-6:1
- Mate:378: din_en_iso_4762_m3x10:24 ↔ mutter_din934_m3-6:3
- Mate:379: Heatsink:1 ↔ mutter_din934_m3-6:3
- Mate:380: din_en_iso_4762_m3x10:2 ↔ mutter_din934_m3-6:2
- Mate:381: Heatsink:1 ↔ mutter_din934_m3-6:2
- Mate:382: din_en_iso_4762_m3x10:28 ↔ mutter_din934_m3-6:4
- Mate:383: Heatsink:1 ↔ mutter_din934_m3-6:4
- Mate:384: GT175DA120U:3 ↔ din_en_iso_4762_m4x6:1
- Mate:385: GT175DA120U:1 ↔ din_en_iso_4762_m4x6:2
- Mate:386: GT175DA120U:2 ↔ din_en_iso_4762_m4x6:3
- Mate:387: IGBT_Platine:2 ↔ din_en_iso_4762_m4x6:3
- Mate:388: IGBT_Platine:3 ↔ din_en_iso_4762_m4x6:1
- Mate:389: IGBT_Platine:1 ↔ din_en_iso_4762_m4x6:2
- Mate:390: GT175DA120U:4 ↔ din_en_iso_4762_m4x6:4
- Mate:391: IGBT_Platine:4 ↔ din_en_iso_4762_m4x6:4
- Mate:392: Heatsink:1 ↔ Cap_Holder_1:2
- Mate:393: CT:2 ↔ CT_Holder:2
- Mate:394: CT:1 ↔ CT_Holder:2
- Flush:15: CT:1 ↔ CT_Holder:2
- Flush:16: CT:2 ↔ CT_Holder:2
- Mate:395: Heatsink:1 ↔ CT_Holder:2
- Mate:396: CT:3 ↔ CT_Holder:1
- Mate:397: CT:4 ↔ CT_Holder:1
- Flush:17: CT:3 ↔ CT_Holder:1
- Flush:18: CT:4 ↔ CT_Holder:1
- Mate:398: Heatsink:1 ↔ CT_Holder:1
- Mate:399: Heatsink:1 ↔ Cap_Holder_1:1
- Mate:400: Heatsink:1 ↔ Cap_Holder_1:1
- Mate:401: Heatsink:1 ↔ Cap_Holder_1:2
- Mate:406: Cap_Holder_1:2 ↔ Cap:2
- Mate:407: Cap_Holder_1:1 ↔ Cap:1
- Mate:412: Abstandshalter_10mm_M4:14 ↔ CU2:1
- Mate:414: Cap:2 ↔ CU2:1
- Mate:415: Cap:1 ↔ CU2:1
- Mate:416: Abstandshalter_10mm_M4:14 ↔ din_en_iso_4762_m4x6:5
- Mate:417: Abstandshalter_10mm_M4:16 ↔ din_en_iso_4762_m4x6:9
- Mate:418: CU2:1 ↔ din_en_iso_4762_m4x6:9
- Mate:419: CU2:1 ↔ din_en_iso_4762_m4x6:5
- Mate:420: Abstandshalter_10mm_M4:6 ↔ din_en_iso_4762_m4x6:8
- Mate:421: Abstandshalter_10mm_M4:7 ↔ din_en_iso_4762_m4x6:6
- Mate:422: Abstandshalter_10mm_M4:5 ↔ din_en_iso_4762_m4x6:7
- Mate:429: Cap:2 ↔ CU4:1
- Mate:430: Cap:2 ↔ CU4:1
- Mate:431: Cap:1 ↔ CU4:1
- Mate:434: Abstandshalter_10mm_M4:4 ↔ CU5:1
- Mate:437: Abstandshalter_10mm_M4:5 ↔ CU5:2
- Mate:438: CU2:1 ↔ Snubber:4
- Mate:439: CU2:1 ↔ Snubber:2
- Mate:440: Abstandshalter_10mm_M4:2 ↔ CU6:1
- Mate:441: Abstandshalter_10mm_M4:1 ↔ CU6:1
- Mate:442: Abstandshalter_10mm_M4:8 ↔ CU6:1
- Mate:443: CU2:1 ↔ din_en_iso_4762_m4x6:5
- Mate:444: CU2:1 ↔ din_en_iso_4762_m4x6:9
- Mate:445: din_en_iso_4762_m4x6:7 ↔ CU5:2
- Mate:446: Snubber:1 ↔ CU6:1
- Mate:447: Snubber:3 ↔ CU6:1
- Mate:449: Snubber:1 ↔ CU6:1
- Mate:450: Abstandshalter_10mm_M4:12 ↔ CU5:1
- Mate:451: Abstandshalter_10mm_M4:4 ↔ CU5:1
- Mate:452: Snubber:3 ↔ CU6:1
